# Autodesk Inventor assembly: Assembly
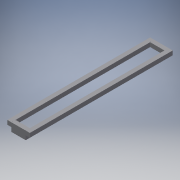
[picture p0: Inventor's stored thumbnail of the model, 180x180]
Saved by Autodesk Inventor 2017 (Build 210142000, 142)
## iProperties
Created: 2019-07-06
Part Number: Assembly
Document SubType Name: Assembly
Designer: Ole Simmering
Author: Ole Simmering
## Documents named in this file (3)
- C:\Users\Ole Simmering\Documents\GitHub\3D_modeling\Guillotine\Assembly.iam
- C:\Users\Ole Simmering\Documents\GitHub\3D_modeling\Guillotine\4ix4ix6i.ipt
- C:\Users\Ole Simmering\Documents\GitHub\3D_modeling\Guillotine\4ix4ix10feet.ipt
## Components (5 placed, 2 different names)
1. 4ix4ix10feet:1 — Mate:2, Flush:3, Flush:4, Mate:3, Flush:5, Flush:6
2. 4ix4ix10feet:2 — Mate:1, Flush:1, Flush:2, Mate:5
3. 4ix4ix6i:1 — Mate:3, Flush:5, Flush:6
4. 4ix4ix6i:2 — Mate:1, Flush:1, Flush:2, Mate:2, Flush:3, Flush:4, Mate:4, Flush:7
5. 4ix4ix6i:5 — Mate:4, Mate:5, Flush:7
## Relationships (12: Flush 7, Mate 5)
- Mate:1: 4ix4ix10feet:2 ↔ 4ix4ix6i:2
- Flush:1: 4ix4ix10feet:2 ↔ 4ix4ix6i:2
- Flush:2: 4ix4ix10feet:2 ↔ 4ix4ix6i:2
- Mate:2: 4ix4ix10feet:1 ↔ 4ix4ix6i:2
- Flush:3: 4ix4ix10feet:1 ↔ 4ix4ix6i:2
- Flush:4: 4ix4ix10feet:1 ↔ 4ix4ix6i:2
- Mate:3: 4ix4ix10feet:1 ↔ 4ix4ix6i:1
- Flush:5: 4ix4ix10feet:1 ↔ 4ix4ix6i:1
- Flush:6: 4ix4ix10feet:1 ↔ 4ix4ix6i:1
- Mate:4: 4ix4ix6i:2 ↔ 4ix4ix6i:5
- Mate:5: 4ix4ix10feet:2 ↔ 4ix4ix6i:5
- Flush:7: 4ix4ix6i:2 ↔ 4ix4ix6i:5
